# Autodesk Inventor assembly: しゃーし
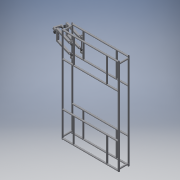
[picture p0: Inventor's stored thumbnail of the model, 180x180]
Saved by Autodesk Inventor 2018 (Build 220112000, 112)
## iProperties
Created: 2017-09-10
Part Number: しゃーし
Material: 一般
Document SubType Name: Assembly
Designer: Kenta
Author: Kenta
## Documents named in this file (8)
- C:\Users\Kenta\Documents\workspace\rbbr\cart\シャーシ\しゃーし.iam
- C:\Users\Kenta\Documents\workspace\rbbr\cart\シャーシ\横のパイプ.ipt
- C:\Users\Kenta\Documents\workspace\rbbr\cart\シャーシ\縦のパイプ.ipt
- C:\Users\Kenta\Documents\workspace\rbbr\cart\シャーシ\高さのパイプ.ipt
- C:\Users\Kenta\Documents\workspace\rbbr\cart\シャーシ\サス付けるパイプ.ipt
- C:\Users\Kenta\Documents\workspace\rbbr\cart\シャーシ\飛び出す奴上.iam
- C:\Users\Kenta\Documents\workspace\rbbr\cart\A.iam
- C:\Users\Kenta\Documents\workspace\rbbr\cart\車輪取り付け部.iam
## Components (29 placed, 7 different names)
1. 横のパイプ:1 — メイト:1, メイト:2, メイト:4, メイト:6, メイト:7, メイト:8, 角度:1, メイト:48, メイト:49
2. 縦のパイプ:1 — メイト:3, メイト:4, メイト:7, メイト:9, メイト:11, メイト:12, メイト:25, メイト:28, メイト:29, フラッシュ:3, メイト:39, メイト:40, メイト:73
3. 縦のパイプ:2 — メイト:5, メイト:6, メイト:8, メイト:10, メイト:21, メイト:23, メイト:27, メイト:30, メイト:41, メイト:42
4. 横のパイプ:2 — メイト:9, メイト:10, メイト:11, メイト:52, メイト:53, メイト:72
5. 高さのパイプ:1 — メイト:12, 角度:1, メイト:20, メイト:28
6. 横のパイプ:3 — メイト:45, メイト:47
7. 縦のパイプ:3 — メイト:20, メイト:24, フラッシュ:3, メイト:35, メイト:36
8. 縦のパイプ:4 — メイト:22, メイト:26, メイト:37, メイト:38
9. 横のパイプ:4 — メイト:50, メイト:51
10. 高さのパイプ:2 — メイト:24, メイト:25, メイト:29
11. 高さのパイプ:3 — メイト:23, メイト:26, メイト:30
12. 高さのパイプ:4 — メイト:21, メイト:22, メイト:27
13. 横のパイプ:5 — メイト:36, メイト:37, メイト:44, メイト:59, メイト:60
14. 横のパイプ:6 — メイト:35, メイト:38, メイト:43, メイト:46, メイト:56
15. 横のパイプ:7 — メイト:40, メイト:42, メイト:44, メイト:57, メイト:58
16. 横のパイプ:8 — メイト:39, メイト:41, メイト:43, メイト:54, メイト:55
17. サス付けるパイプ:1 — メイト:45, メイト:46, メイト:62
18. サス付けるパイプ:2 — メイト:48, メイト:55, メイト:61
19. サス付けるパイプ:3 — メイト:49, メイト:54, メイト:62
20. サス付けるパイプ:4 — メイト:47, メイト:56, メイト:61
21. サス付けるパイプ:5 — メイト:50, メイト:59, メイト:64
22. サス付けるパイプ:6 — メイト:53, メイト:58, メイト:64
23. サス付けるパイプ:7 — メイト:52, メイト:57, メイト:63, メイト:68, メイト:73
24. サス付けるパイプ:8 — メイト:51, メイト:60, メイト:63, メイト:66
25. 飛び出す奴上:1 [sub-assembly] — 角度:5, メイト:66, フラッシュ:4, メイト:74, メイト:76
26. 飛び出す奴上:3 [sub-assembly] — 角度:3, メイト:68, フラッシュ:4, メイト:72, メイト:75
27. A:1 [sub-assembly] — メイト:74, フラッシュ:5, 角度:6, メイト:76, 回転:1
28. A:2 [sub-assembly] — メイト:75, フラッシュ:5, 角度:6
29. 車輪取り付け部:1 [sub-assembly] — 回転:1
## Relationships (77: Mate 67, Flush 5, Angle 4, RevoluteJoint 1)
- フラッシュ:1 [Flush]
- メイト:1 [Mate]: 横のパイプ:1
- フラッシュ:2 [Flush]
- メイト:2 [Mate]: 横のパイプ:1
- メイト:3 [Mate]: 縦のパイプ:1
- メイト:4 [Mate]: 横のパイプ:1 ↔ 縦のパイプ:1
- メイト:5 [Mate]: 縦のパイプ:2
- メイト:6 [Mate]: 横のパイプ:1 ↔ 縦のパイプ:2
- メイト:7 [Mate] (-13.6 mm): 横のパイプ:1 ↔ 縦のパイプ:1
- メイト:8 [Mate] (-13.6 mm): 横のパイプ:1 ↔ 縦のパイプ:2
- メイト:9 [Mate]: 縦のパイプ:1 ↔ 横のパイプ:2
- メイト:10 [Mate]: 縦のパイプ:2 ↔ 横のパイプ:2
- メイト:11 [Mate] (-13.6 mm): 縦のパイプ:1 ↔ 横のパイプ:2
- メイト:12 [Mate]: 縦のパイプ:1 ↔ 高さのパイプ:1
- 角度:1 [Angle] (-90 deg): 横のパイプ:1 ↔ 高さのパイプ:1
- [Mate]: 横のパイプ:3 ↔ 縦のパイプ:3
- [Mate]: 横のパイプ:3 ↔ 縦のパイプ:4
- [Mate] (-13.6 mm): 横のパイプ:3 ↔ 縦のパイプ:3
- [Mate] (-13.6 mm): 横のパイプ:3 ↔ 縦のパイプ:4
- [Mate]: 縦のパイプ:3 ↔ 横のパイプ:4
- [Mate]: 縦のパイプ:4 ↔ 横のパイプ:4
- [Mate] (-13.6 mm): 縦のパイプ:3 ↔ 横のパイプ:4
- メイト:20 [Mate]: 高さのパイプ:1 ↔ 縦のパイプ:3
- メイト:21 [Mate]: 縦のパイプ:2 ↔ 高さのパイプ:4
- メイト:22 [Mate]: 縦のパイプ:4 ↔ 高さのパイプ:4
- メイト:23 [Mate]: 縦のパイプ:2 ↔ 高さのパイプ:3
- メイト:24 [Mate]: 縦のパイプ:3 ↔ 高さのパイプ:2
- メイト:25 [Mate]: 縦のパイプ:1 ↔ 高さのパイプ:2
- メイト:26 [Mate]: 縦のパイプ:4 ↔ 高さのパイプ:3
- メイト:27 [Mate] (-40.8 mm): 縦のパイプ:2 ↔ 高さのパイプ:4
- メイト:28 [Mate] (-40.8 mm): 縦のパイプ:1 ↔ 高さのパイプ:1
- メイト:29 [Mate] (-40.8 mm): 縦のパイプ:1 ↔ 高さのパイプ:2
- メイト:30 [Mate] (-40.8 mm): 縦のパイプ:2 ↔ 高さのパイプ:3
- フラッシュ:3 [Flush]: 縦のパイプ:1 ↔ 縦のパイプ:3
- メイト:35 [Mate]: 縦のパイプ:3 ↔ 横のパイプ:6
- メイト:36 [Mate]: 縦のパイプ:3 ↔ 横のパイプ:5
- メイト:37 [Mate]: 縦のパイプ:4 ↔ 横のパイプ:5
- メイト:38 [Mate]: 縦のパイプ:4 ↔ 横のパイプ:6
- メイト:39 [Mate]: 縦のパイプ:1 ↔ 横のパイプ:8
- メイト:40 [Mate]: 縦のパイプ:1 ↔ 横のパイプ:7
- メイト:41 [Mate]: 縦のパイプ:2 ↔ 横のパイプ:8
- メイト:42 [Mate]: 縦のパイプ:2 ↔ 横のパイプ:7
- メイト:43 [Mate]: 横のパイプ:6 ↔ 横のパイプ:8
- メイト:44 [Mate]: 横のパイプ:5 ↔ 横のパイプ:7
- メイト:45 [Mate]: 横のパイプ:3 ↔ サス付けるパイプ:1
- メイト:46 [Mate]: 横のパイプ:6 ↔ サス付けるパイプ:1
- メイト:47 [Mate]: 横のパイプ:3 ↔ サス付けるパイプ:4
- メイト:48 [Mate]: 横のパイプ:1 ↔ サス付けるパイプ:2
- メイト:49 [Mate]: 横のパイプ:1 ↔ サス付けるパイプ:3
- メイト:50 [Mate]: 横のパイプ:4 ↔ サス付けるパイプ:5
- メイト:51 [Mate]: 横のパイプ:4 ↔ サス付けるパイプ:8
- メイト:52 [Mate]: 横のパイプ:2 ↔ サス付けるパイプ:7
- メイト:53 [Mate]: 横のパイプ:2 ↔ サス付けるパイプ:6
- メイト:54 [Mate]: 横のパイプ:8 ↔ サス付けるパイプ:3
- メイト:55 [Mate]: 横のパイプ:8 ↔ サス付けるパイプ:2
- メイト:56 [Mate]: 横のパイプ:6 ↔ サス付けるパイプ:4
- メイト:57 [Mate]: 横のパイプ:7 ↔ サス付けるパイプ:7
- メイト:58 [Mate]: 横のパイプ:7 ↔ サス付けるパイプ:6
- メイト:59 [Mate]: 横のパイプ:5 ↔ サス付けるパイプ:5
- メイト:60 [Mate]: 横のパイプ:5 ↔ サス付けるパイプ:8
- メイト:61 [Mate]: サス付けるパイプ:2 ↔ サス付けるパイプ:4
- メイト:62 [Mate]: サス付けるパイプ:1 ↔ サス付けるパイプ:3
- メイト:63 [Mate]: サス付けるパイプ:7 ↔ サス付けるパイプ:8
- メイト:64 [Mate]: サス付けるパイプ:5 ↔ サス付けるパイプ:6
- 角度:3 [Angle] (0 deg): 飛び出す奴上:3
- 角度:5 [Angle] (0 deg): 飛び出す奴上:1
- メイト:66 [Mate]: サス付けるパイプ:8 ↔ 飛び出す奴上:1
- メイト:68 [Mate]: サス付けるパイプ:7 ↔ 飛び出す奴上:3
- フラッシュ:4 [Flush]: 飛び出す奴上:1 ↔ 飛び出す奴上:3
- メイト:72 [Mate] (100 mm): 横のパイプ:2 ↔ 飛び出す奴上:3
- メイト:73 [Mate] (200 mm): 縦のパイプ:1 ↔ サス付けるパイプ:7
- メイト:74 [Mate]: 飛び出す奴上:1 ↔ A:1
- メイト:75 [Mate]: 飛び出す奴上:3 ↔ A:2
- フラッシュ:5 [Flush]: A:1 ↔ A:2
- 角度:6 [Angle] (0 deg): A:1 ↔ A:2
- メイト:76 [Mate] (5 mm): 飛び出す奴上:1 ↔ A:1
- 回転:1 [RevoluteJoint]: A:1 ↔ 車輪取り付け部:1
## Named parameters: d21_d13 = 0 mm, d22_d15 = 0 mm, d23_d16 = -13.6 mm, d24_d8 = 0 mm, d25_d10 = 0 mm, d26_d11 = -13.6 mm, d27_d12 = -13.6 mm
